# Autodesk Inventor assembly: Assembly
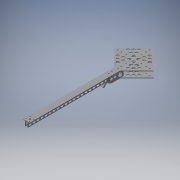
[picture p0: Inventor's stored thumbnail of the model, 180x180]
Saved by Autodesk Inventor 2016 (Build 200138000, 138)
## iProperties
Created: 2016-03-06
Part Number: Assembly
Document SubType Name: Assembly
Designer: dimas
Author: dimas
## Documents named in this file (4)
- C:\Users\dimas\Documents\lap_quad\Assembly.iam
- C:\Users\dimas\Documents\lap_quad\Arm_light.ipt
- C:\Users\dimas\Documents\lap_quad\frame_mount.ipt
- C:\Users\dimas\Documents\lap_quad\plate_mk2.ipt
## Components (4 placed, 3 different names)
1. Arm_light:1 — Mate:1, Mate:2, Flush:1
2. frame_mount:1 — Mate:1, Mate:2, Flush:1, Mate:3, Mate:4, Flush:2, Mate:5, Mate:6, Flush:3
3. plate_mk2:1 — Mate:3, Mate:4, Flush:2
4. plate_mk2:2 — Mate:5, Mate:6, Flush:3
## Relationships (9: Mate 6, Flush 3)
- Mate:1: Arm_light:1 ↔ frame_mount:1
- Mate:2: Arm_light:1 ↔ frame_mount:1
- Flush:1: Arm_light:1 ↔ frame_mount:1
- Mate:3: frame_mount:1 ↔ plate_mk2:1
- Mate:4: frame_mount:1 ↔ plate_mk2:1
- Flush:2: frame_mount:1 ↔ plate_mk2:1
- Mate:5: frame_mount:1 ↔ plate_mk2:2
- Mate:6: frame_mount:1 ↔ plate_mk2:2
- Flush:3: frame_mount:1 ↔ plate_mk2:2
